# Autodesk Inventor assembly: Сборка4
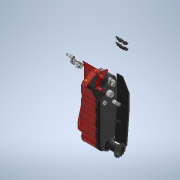
[picture p0: Inventor's stored thumbnail of the model, 180x180]
Saved by Autodesk Inventor 2020 (Build 240168000, 168)
## iProperties
Created: 2021-02-19
Part Number: Сборка4
Document SubType Name: Assembly
Designer: Pariah
Author: Pariah
## Documents named in this file (39)
- C:\Users\I_Love_U_Bogdan\Desktop\Work\Гусеничная платформа\Сборка4.iam
- C:\Users\I_Love_U_Bogdan\Desktop\Work\Гусеничная платформа\Корпус.ipt
- C:\Users\I_Love_U_Bogdan\Desktop\Work\Гусеничная платформа\Крышка.ipt
- C:\Users\I_Love_U_Bogdan\Desktop\Work\Гусеничная платформа\Перед-верх.ipt
- C:\Users\I_Love_U_Bogdan\Desktop\Work\Гусеничная платформа\Потшипник 22-8.ipt
- C:\Users\I_Love_U_Bogdan\Desktop\Work\Гусеничная платформа\СкреплениеКорпусПеред.ipt
- C:\Users\I_Love_U_Bogdan\Desktop\Work\Гусеничная платформа\РеброСкрепления.ipt
- C:\Users\I_Love_U_Bogdan\Desktop\Work\Гусеничная платформа\Трак.ipt
- C:\Users\I_Love_U_Bogdan\Desktop\Work\Гусеничная платформа\ОпорныйКаток2.ipt
- C:\Users\I_Love_U_Bogdan\Desktop\Work\ПечатьДом\Шаговик17.ipt
- C:\Users\I_Love_U_Bogdan\Desktop\Work\Гусеничная платформа\Муфта2.ipt
- C:\Users\I_Love_U_Bogdan\Desktop\Work\Гусеничная платформа\РычагОпорного.ipt
- C:\Users\I_Love_U_Bogdan\Desktop\Work\Гусеничная платформа\ОпорныйКаток.ipt
- C:\Users\I_Love_U_Bogdan\Desktop\Work\Гусеничная платформа\Корпус внутр.ipt
- C:\Users\I_Love_U_Bogdan\Desktop\Work\Гусеничная платформа\Корпус внутр2.ipt
- C:\Users\I_Love_U_Bogdan\Desktop\Work\Гусеничная платформа\Корпус4.ipt
- C:\Users\I_Love_U_Bogdan\Desktop\Work\ПечатьДом\Крепление плат.ipt
- C:\Users\I_Love_U_Bogdan\Desktop\Work\Гусеничная платформа\Зажим проводов.ipt
- C:\Users\I_Love_U_Bogdan\Desktop\Work\Гусеничная платформа\ВедущееКолесо V2.ipt
- C:\Users\I_Love_U_Bogdan\Desktop\Work\Гусеничная платформа\Втулка.ipt
- C:\Users\I_Love_U_Bogdan\Desktop\Work\Гусеничная платформа\ВнутрНат.ipt
- C:\Users\I_Love_U_Bogdan\Desktop\Work\Гусеничная платформа\ВнешНат.ipt
- C:\Users\I_Love_U_Bogdan\Desktop\Work\Гусеничная платформа\ВнутрНатПр.ipt
- C:\Users\I_Love_U_Bogdan\Desktop\Work\Гусеничная платформа\ВнешНатПр.ipt
- C:\Users\I_Love_U_Bogdan\Desktop\Work\Гусеничная платформа\Пластина.ipt
- C:\Users\I_Love_U_Bogdan\Desktop\Work\Гусеничная платформа\Шаблон.ipt
- C:\Users\I_Love_U_Bogdan\Desktop\Work\Гусеничная платформа\Подпорный.ipt
- C:\Users\I_Love_U_Bogdan\Desktop\Work\Гусеничная платформа\Потшипник.ipt
- C:\Users\I_Love_U_Bogdan\Desktop\Work\Гусеничная платформа\ПодпорныйКаток.ipt
- C:\Users\I_Love_U_Bogdan\Desktop\Work\Гусеничная платформа\запорные зубцы.ipt
- C:\Users\I_Love_U_Bogdan\Desktop\Work\Гусеничная платформа\Держатель каскада.ipt
- C:\Users\I_Love_U_Bogdan\Desktop\Work\Гусеничная платформа\РучкаКрышки.ipt
- C:\Users\I_Love_U_Bogdan\Desktop\Work\Гусеничная платформа\РельсКрышки.ipt
- C:\Users\I_Love_U_Bogdan\Desktop\Work\Гусеничная платформа\Шаблон2.ipt
- C:\Users\I_Love_U_Bogdan\Desktop\Work\Гусеничная платформа\Печать\Надкрылок.ipt
- C:\Users\I_Love_U_Bogdan\Desktop\Work\Гусеничная платформа\ВерхнийКрюк.ipt
- C:\Users\I_Love_U_Bogdan\Desktop\Work\Гусеничная платформа\Крепление лидара.ipt
- C:\Users\I_Love_U_Bogdan\Desktop\Work\Гусеничная платформа\Чаша1.ipt
- C:\Users\I_Love_U_Bogdan\Desktop\Work\Гусеничная платформа\ТракV2.ipt
## Components (49 placed, 38 different names)
1. Шаговик17:1 — Совмещение:50, Совмещение:51, Совмещение:52, Совмещение:58
2. Потшипник 22-8:1 — Вставка:1
3. Трак:1 — Совмещение:64, Заподлицо:42, Заподлицо:43
4. ОпорныйКаток2:2
5. РычагОпорного:1 — Совмещение:43, Совмещение:45, Совмещение:46
6. ОпорныйКаток2:3 — Совмещение:45, Совмещение:46, Заподлицо:18
7. ОпорныйКаток:1
8. ОпорныйКаток2:4 — Заподлицо:18
9. Крепление плат:1 — Заподлицо:21, Совмещение:55, Совмещение:56
10. Зажим проводов:1 — Заподлицо:21
11. Шаблон:1 — Заподлицо:27, Заподлицо:28
12. Подпорный:1 — Заподлицо:29, Заподлицо:30
13. Потшипник:1 — Заподлицо:30, Заподлицо:31, Заподлицо:32
14. ПодпорныйКаток:1 — Заподлицо:31, Заподлицо:32
15. РельсКрышки:1 — Заподлицо:36
16. Шаблон2:1 — Заподлицо:37
17. Надкрылок:1 — Заподлицо:38
18. ВерхнийКрюк:1 — Заподлицо:39
19. Крепление лидара:1 — Заподлицо:40, Заподлицо:41
20. Чаша1:1 — Заподлицо:41
21. ТракV2:1 — Заподлицо:42, Заподлицо:43
22. Левый1 — Совмещение:1, Совмещение:4, Совмещение:5, Заподлицо:1, Вставка:1, Совмещение:7, Совмещение:8, Совмещение:9, Совмещение:10, Совмещение:11, Совмещение:12, Совмещение:13, Совмещение:14, Совмещение:15, Совмещение:16, Совмещение:17, Совмещение:18, Совмещение:19, Совмещение:20, Совмещение:43, Совмещение:50, Совмещение:51, Совмещение:52, Совмещение:53, Заподлицо:19, Заподлицо:20, Совмещение:59, Заподлицо:22, Заподлицо:27, Заподлицо:28, Заподлицо:29, Совмещение:64, Заподлицо:36, Заподлицо:37, Заподлицо:38
23. Левый2 — Совмещение:53, Заподлицо:19, Заподлицо:20, Совмещение:55
24. Правый2
25. Правый1 — Совмещение:56
26. Перед-верх:1 — Совмещение:4, Совмещение:5, Заподлицо:1, Совмещение:6, Заподлицо:2, Заподлицо:33, Заподлицо:39, Заподлицо:40
27. СкреплениеКорпусПеред:1 — Совмещение:19, Совмещение:20
28. РеброСкрепления:1
29. РеброСкрепления:2 — Совмещение:7, Совмещение:8, Совмещение:9
30. РеброСкрепления:3 — Совмещение:10, Совмещение:14, Совмещение:16
31. РеброСкрепления:4 — Совмещение:11, Совмещение:13, Совмещение:17
32. РеброСкрепления:5 — Совмещение:12, Совмещение:15, Совмещение:18
33. ВедущееКолесо V2:1 — Совмещение:58, Совмещение:59, Совмещение:62, Совмещение:63
34. Муфта2:1 — Совмещение:62, Совмещение:63
35. Втулка:1 — Заподлицо:22, Совмещение:60, Совмещение:61
36. ВнутрНат:1 — Совмещение:60, Совмещение:61, Заподлицо:23, Заподлицо:24
37. ВнешНат:1 — Заподлицо:23, Заподлицо:24
38. ВнутрНатПр:1
39. ВнешНатПр:1
40. РучкаКрышки:1 — Заподлицо:35
41. Держатель каскада:1 — Заподлицо:34
42. запорные зубцы:1 — Заподлицо:33
43. Крышка:1 — Совмещение:1, Совмещение:6, Заподлицо:2, Заподлицо:25, Заподлицо:26, Заподлицо:34, Заподлицо:35
44. Пластина:1 — Заподлицо:25, Заподлицо:26
45. Пластина:2
46. Пластина:3
47. Пластина:4
48. Пластина:5
49. Пластина:6
## Component patterns: (6 elements, first: Пластина:1)
## Relationships (63: Mate 34, Flush 28, Insert 1)
- Совмещение:1 [Mate] (0.2 mm): Левый1 ↔ Крышка:1
- Совмещение:4 [Mate] (0.1 mm): Левый1 ↔ Перед-верх:1
- Совмещение:5 [Mate]: Левый1 ↔ Перед-верх:1
- Заподлицо:1 [Flush]: Левый1 ↔ Перед-верх:1
- Вставка:1 [Insert] (-8.8 mm): Потшипник 22-8:1 ↔ Левый1
- Совмещение:6 [Mate] (0.1 mm): Перед-верх:1 ↔ Крышка:1
- Заподлицо:2 [Flush]: Перед-верх:1 ↔ Крышка:1
- Совмещение:7 [Mate]: Левый1 ↔ РеброСкрепления:2
- Совмещение:8 [Mate] (0.1 mm): Левый1 ↔ РеброСкрепления:2
- Совмещение:9 [Mate] (0.1 mm): Левый1 ↔ РеброСкрепления:2
- Совмещение:10 [Mate]: Левый1 ↔ РеброСкрепления:3
- Совмещение:11 [Mate]: Левый1 ↔ РеброСкрепления:4
- Совмещение:12 [Mate]: Левый1 ↔ РеброСкрепления:5
- Совмещение:13 [Mate] (0.1 mm): Левый1 ↔ РеброСкрепления:4
- Совмещение:14 [Mate] (0.1 mm): Левый1 ↔ РеброСкрепления:3
- Совмещение:15 [Mate] (0.1 mm): Левый1 ↔ РеброСкрепления:5
- Совмещение:16 [Mate] (0.1 mm): Левый1 ↔ РеброСкрепления:3
- Совмещение:17 [Mate] (0.1 mm): Левый1 ↔ РеброСкрепления:4
- Совмещение:18 [Mate] (0.1 mm): Левый1 ↔ РеброСкрепления:5
- Совмещение:19 [Mate]: Левый1 ↔ СкреплениеКорпусПеред:1
- Совмещение:20 [Mate]: Левый1 ↔ СкреплениеКорпусПеред:1
- Совмещение:43 [Mate] (2 mm): РычагОпорного:1 ↔ Левый1
- Совмещение:45 [Mate]: РычагОпорного:1 ↔ ОпорныйКаток2:3
- Совмещение:46 [Mate] (0.2 mm): РычагОпорного:1 ↔ ОпорныйКаток2:3
- Заподлицо:18 [Flush]: ОпорныйКаток2:3 ↔ ОпорныйКаток2:4
- Совмещение:50 [Mate] (1.5 mm): Шаговик17:1 ↔ Левый1
- Совмещение:51 [Mate]: Шаговик17:1 ↔ Левый1
- Совмещение:52 [Mate] (4 mm): Шаговик17:1 ↔ Левый1
- Совмещение:53 [Mate]: Левый1 ↔ Левый2
- Заподлицо:19 [Flush]: Левый1 ↔ Левый2
- Заподлицо:20 [Flush]: Левый1 ↔ Левый2
- Заподлицо:21 [Flush]: Крепление плат:1 ↔ Зажим проводов:1
- Совмещение:55 [Mate] (20 mm): Крепление плат:1 ↔ Левый2
- Совмещение:56 [Mate] (11 mm): Крепление плат:1 ↔ Правый1
- Совмещение:58 [Mate]: Шаговик17:1 ↔ ВедущееКолесо V2:1
- Совмещение:59 [Mate] (2 mm): Левый1 ↔ ВедущееКолесо V2:1
- Заподлицо:22 [Flush]: Левый1 ↔ Втулка:1
- Совмещение:60 [Mate]: Втулка:1 ↔ ВнутрНат:1
- Совмещение:61 [Mate] (0.1 mm): Втулка:1 ↔ ВнутрНат:1
- Заподлицо:23 [Flush]: ВнутрНат:1 ↔ ВнешНат:1
- Заподлицо:24 [Flush]: ВнутрНат:1 ↔ ВнешНат:1
- Заподлицо:25 [Flush]: Крышка:1 ↔ Пластина:1
- Заподлицо:26 [Flush]: Крышка:1 ↔ Пластина:1
- Заподлицо:27 [Flush]: Шаблон:1 ↔ Левый1
- Заподлицо:28 [Flush]: Шаблон:1 ↔ Левый1
- Совмещение:62 [Mate]: ВедущееКолесо V2:1 ↔ Муфта2:1
- Совмещение:63 [Mate] (0.2 mm): ВедущееКолесо V2:1 ↔ Муфта2:1
- Заподлицо:29 [Flush]: Подпорный:1 ↔ Левый1
- Совмещение:64 [Mate] (8 mm): Трак:1 ↔ Левый1
- Заподлицо:30 [Flush]: Подпорный:1 ↔ Потшипник:1
- Заподлицо:31 [Flush]: Потшипник:1 ↔ ПодпорныйКаток:1
- Заподлицо:32 [Flush]: Потшипник:1 ↔ ПодпорныйКаток:1
- Заподлицо:33 [Flush]: Перед-верх:1 ↔ запорные зубцы:1
- Заподлицо:34 [Flush]: Держатель каскада:1 ↔ Крышка:1
- Заподлицо:35 [Flush]: РучкаКрышки:1 ↔ Крышка:1
- Заподлицо:36 [Flush]: РельсКрышки:1 ↔ Левый1
- Заподлицо:37 [Flush]: Шаблон2:1 ↔ Левый1
- Заподлицо:38 [Flush]: Надкрылок:1 ↔ Левый1
- Заподлицо:39 [Flush]: ВерхнийКрюк:1 ↔ Перед-верх:1
- Заподлицо:40 [Flush]: Крепление лидара:1 ↔ Перед-верх:1
- Заподлицо:41 [Flush]: Крепление лидара:1 ↔ Чаша1:1
- Заподлицо:42 [Flush]: Трак:1 ↔ ТракV2:1
- Заподлицо:43 [Flush]: Трак:1 ↔ ТракV2:1
